# Autodesk Inventor assembly: DriveTrainWelding_20Jan
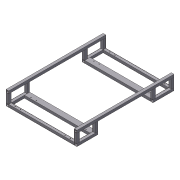
[picture p0: Inventor's stored thumbnail of the model, 180x180]
Saved by Autodesk Inventor 2012 (Build 160160000, 160)
## iProperties
Created: 2012-01-20
Part Number: DriveTrainWelding_20Jan
Document SubType Name: Assembly
Designer: JesseK
Author: JesseK
## Documents named in this file (3)
- Z:\UserData\Documents\Inventor\team1885frc\Robot2012\Drawings\DriveTrainWelding_20Jan.iam
- Z:\UserData\Documents\Inventor\team1885frc\Robot2012\Drawings\CrossBarAssembly.iam
- Z:\UserData\Documents\Inventor\team1885frc\Robot2012\Drawings\WheelPod_ForDrawing.iam
## Components (4 placed, 2 different names)
1. CrossBarAssembly:1 [sub-assembly] — Flush:1, Flush:2, Mate:2, Flush:5, Mate:3, Mate:4
2. CrossBarAssembly:2 [sub-assembly] — Flush:3, Flush:4, Mate:1
3. WheelPod_ForDrawing:1 [sub-assembly] — Flush:1, Flush:2, Flush:3, Flush:4, Mate:1, Mate:2
4. WheelPod_ForDrawing:2 [sub-assembly] — Flush:5, Mate:3, Mate:4
## Relationships (9: Flush 5, Mate 4)
- Flush:1: CrossBarAssembly:1 ↔ WheelPod_ForDrawing:1
- Flush:2: CrossBarAssembly:1 ↔ WheelPod_ForDrawing:1
- Flush:3: CrossBarAssembly:2 ↔ WheelPod_ForDrawing:1
- Flush:4: CrossBarAssembly:2 ↔ WheelPod_ForDrawing:1
- Mate:1: CrossBarAssembly:2 ↔ WheelPod_ForDrawing:1
- Mate:2: CrossBarAssembly:1 ↔ WheelPod_ForDrawing:1
- Flush:5: CrossBarAssembly:1 ↔ WheelPod_ForDrawing:2
- Mate:3: CrossBarAssembly:1 ↔ WheelPod_ForDrawing:2
- Mate:4: CrossBarAssembly:1 ↔ WheelPod_ForDrawing:2
